# Autodesk Inventor assembly: A105EnsembleBoitierLaserV2
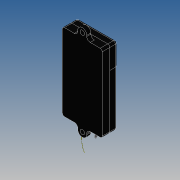
[picture p0: Inventor's stored thumbnail of the model, 180x180]
Saved by Autodesk Inventor 2019 (Build 230136000, 136)
## iProperties
Created: 2017-01-30
Part Number: A105EnsembleBoitierLaserV2
Document SubType Name: Assembly
Designer: serge.amoos
Author: serge.amoos
## Documents named in this file (13)
- Y:\serge.amoos\AAA-FichiersTries\FocalMeasure\A104EnsembleBoitierLaser.iam
- Y:\serge.amoos\AAA-FichiersTries\FocalMeasure\F111Batterie9V.ipt
- Y:\serge.amoos\AAA-FichiersTries\FocalMeasure\F113PriseBatterie.ipt
- Y:\serge.amoos\AAA-FichiersTries\FocalMeasure\P121BoardLaser.ipt
- Y:\serge.amoos\AAA-FichiersTries\FocalMeasure\F110LaserLP450.iam
- Y:\serge.amoos\AAA-FichiersTries\FocalMeasure\F112Interrupteur.ipt
- Y:\serge.amoos\AAA-FichiersTries\FocalMeasure\P125BoitierFond.ipt
- Y:\serge.amoos\AAA-FichiersTries\FocalMeasure\P126Radiateur.ipt
- Y:\serge.amoos\AAA-FichiersTries\FocalMeasure\P127CouvercleLaser.ipt
- Y:\serge.amoos\AAA-FichiersTries\FocalMeasure\P128CouvercleBatterie.ipt
- Y:\serge.amoos\AAA-FichiersTries\FocalMeasure\P129SigneLaser.ipt
- Y:\serge.amoos\AAA-FichiersTries\FocalMeasure\P130PlaqueLogo.ipt
- Y:\serge.amoos\AAA-FichiersTries\FocalMeasure\P131PlaqueThorlabs.ipt
## Components (12 placed, 12 different names)
1. P125BoitierFond:1 — Mate:3, Mate:6, Mate:7, Mate:9, Mate:10, Mate:11, Insert:2, Angle:3, Mate:12, Mate:13, Mate:14, Mate:15, Flush:1, Mate:16, Flush:2, Mate:18
2. F111Batterie9V:1 — Mate:1, Angle:1, Mate:2, Mate:3, Mate:12, Mate:13
3. F113PriseBatterie:1 — Mate:1, Angle:1, Mate:2
4. P121BoardLaser:1 — Mate:6, Mate:11, Mate:18
5. P126Radiateur:1 — Mate:7, Mate:9, Insert:1, Angle:2, Mate:10
6. F110LaserLP450:1 [sub-assembly] — Insert:1, Angle:2
7. F112Interrupteur:1 — Insert:2, Angle:3
8. P127CouvercleLaser:1 — Mate:14, Mate:15, Flush:1, Mate:17, Mate:19, Mate:20, Mate:21, Mate:22, Mate:23, Mate:24
9. P128CouvercleBatterie:1 — Mate:16, Flush:2, Mate:17
10. P129SigneLaser:1 — Mate:19
11. P130PlaqueLogo:1 — Mate:20, Mate:21, Mate:22
12. P131PlaqueThorlabs:1 — Mate:23, Mate:24
## Relationships (28: Mate 21, Angle 3, Insert 2, Flush 2)
- Mate:1: F111Batterie9V:1 ↔ F113PriseBatterie:1
- Angle:1 (0 deg): F111Batterie9V:1 ↔ F113PriseBatterie:1
- Mate:2 (2.5 mm): F111Batterie9V:1 ↔ F113PriseBatterie:1
- Mate:3: P125BoitierFond:1 ↔ F111Batterie9V:1
- Mate:6 (2 mm): P125BoitierFond:1 ↔ P121BoardLaser:1
- Mate:7: P125BoitierFond:1 ↔ P126Radiateur:1
- Mate:9: P125BoitierFond:1 ↔ P126Radiateur:1
- Insert:1: P126Radiateur:1 ↔ F110LaserLP450:1
- Angle:2 (90 deg): P126Radiateur:1 ↔ F110LaserLP450:1
- Mate:10 (0.1 mm): P125BoitierFond:1 ↔ P126Radiateur:1
- Mate:11 (2 mm): P125BoitierFond:1 ↔ P121BoardLaser:1
- Insert:2: P125BoitierFond:1 ↔ F112Interrupteur:1
- Angle:3 (0 deg): P125BoitierFond:1 ↔ F112Interrupteur:1
- Mate:12 (2 mm): P125BoitierFond:1 ↔ F111Batterie9V:1
- Mate:13 (1 mm): P125BoitierFond:1 ↔ F111Batterie9V:1
- Mate:14: P125BoitierFond:1 ↔ P127CouvercleLaser:1
- Mate:15: P125BoitierFond:1 ↔ P127CouvercleLaser:1
- Flush:1: P125BoitierFond:1 ↔ P127CouvercleLaser:1
- Mate:16: P125BoitierFond:1 ↔ P128CouvercleBatterie:1
- Flush:2: P125BoitierFond:1 ↔ P128CouvercleBatterie:1
- Mate:17: P127CouvercleLaser:1 ↔ P128CouvercleBatterie:1
- Mate:18 (2 mm): P125BoitierFond:1 ↔ P121BoardLaser:1
- Mate:19: P127CouvercleLaser:1 ↔ P129SigneLaser:1
- Mate:20: P127CouvercleLaser:1 ↔ P130PlaqueLogo:1
- Mate:21 (0.2 mm): P127CouvercleLaser:1 ↔ P130PlaqueLogo:1
- Mate:22 (0.2 mm): P127CouvercleLaser:1 ↔ P130PlaqueLogo:1
- Mate:23: P127CouvercleLaser:1 ↔ P131PlaqueThorlabs:1
- Mate:24: P127CouvercleLaser:1 ↔ P131PlaqueThorlabs:1
